# Autodesk Inventor assembly: Assieme2
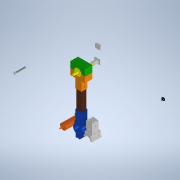
[picture p0: Inventor's stored thumbnail of the model, 180x180]
Saved by Autodesk Inventor 2020 (Build 240168000, 168)
## iProperties
Created: 2019-10-11
Part Number: Assieme2
Document SubType Name: Assembly
Designer: socci
Author: socci
## Documents named in this file (12)
- C:\Users\socci\Desktop\mv-Project\04_PartDraw\Modello_3D.iam
- C:\Users\socci\Desktop\mv-Project\04_PartDraw\Componenti\1_Asse_cuscinetti.ipt
- C:\Users\socci\Desktop\mv-Project\04_PartDraw\Componenti\2_Connettore_inf_sup.ipt
- C:\Users\socci\Desktop\mv-Project\04_PartDraw\Componenti\3_Connettore_inf_INF.ipt
- C:\Users\socci\Desktop\mv-Project\04_PartDraw\Componenti\4_barra.ipt
- C:\Users\socci\Desktop\mv-Project\04_PartDraw\Componenti\5_Connettore_sup_inf.ipt
- C:\Users\socci\Desktop\mv-Project\04_PartDraw\Componenti\6_Vite_M5_L40.ipt
- C:\Users\socci\Desktop\mv-Project\04_PartDraw\Componenti\7_Motore.ipt
- C:\Users\socci\Desktop\mv-Project\04_PartDraw\Componenti\8_Connettore_sup.ipt
- C:\Users\socci\Desktop\mv-Project\04_PartDraw\Componenti\9_Flangia.ipt
- C:\Users\socci\Desktop\mv-Project\04_PartDraw\Componenti\10_MPU_6050.ipt
- C:\Users\socci\Desktop\mv-Project\04_PartDraw\Componenti\11_Connettore_MPU.ipt
## Components (11 placed, 11 different names)
1. 1_Asse_cuscinetti:1 — Inserimento:1, Inserimento:2, Inserimento:3
2. 2_Connettore_inf_sup:1 — Inserimento:1, Coincidente:6, Coincidente:7, Coincidente:8
3. 3_Connettore_inf_INF:1 — Inserimento:2
4. 4_barra:1 — Coincidente:6, Coincidente:7, Coincidente:8, Coincidente:9, Coincidente:10, Coincidente:11
5. 5_Connettore_sup_inf:1 — Coincidente:9, Coincidente:10, Coincidente:11
6. 6_Vite_M5_L40:1
7. 7_Motore:1
8. 8_Connettore_sup:1
9. 9_Flangia:1
10. 10_MPU_6050:1
11. 11_Connettore_MPU:1 — Inserimento:3
## Relationships (9: Mate 6, Insert 3)
- Inserimento:1: 1_Asse_cuscinetti:1 ↔ 2_Connettore_inf_sup:1
- Inserimento:2: 1_Asse_cuscinetti:1 ↔ 3_Connettore_inf_INF:1
- Coincidente:6 [Mate]: 2_Connettore_inf_sup:1 ↔ 4_barra:1
- Coincidente:7 [Mate]: 2_Connettore_inf_sup:1 ↔ 4_barra:1
- Coincidente:8 [Mate]: 2_Connettore_inf_sup:1 ↔ 4_barra:1
- Coincidente:9 [Mate]: 4_barra:1 ↔ 5_Connettore_sup_inf:1
- Coincidente:10 [Mate]: 4_barra:1 ↔ 5_Connettore_sup_inf:1
- Coincidente:11 [Mate]: 4_barra:1 ↔ 5_Connettore_sup_inf:1
- Inserimento:3: 1_Asse_cuscinetti:1 ↔ 11_Connettore_MPU:1
